# Autodesk Inventor assembly: Long Arm
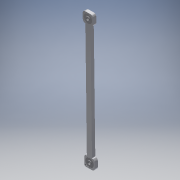
[picture p0: Inventor's stored thumbnail of the model, 180x180]
Saved by Autodesk Inventor 2016 (Build 200138000, 138)
## iProperties
Created: 2015-06-08
Part Number: Long Arm
Document SubType Name: Assembly
Designer: Dennis
Author: Dennis
## Documents named in this file (3)
- C:\Users\Dennis\Dropbox\NI Work\NI Slider Crank\Assemblies\Long Arm.iam
- C:\Users\Dennis\Dropbox\NI Work\NI Slider Crank\Parts\Arm Long.ipt
- C:\Users\Dennis\Dropbox\NI Work\NI Slider Crank\Parts\Bearing - 6384K342.ipt
## Components (3 placed, 2 different names)
1. Arm Long:1 — Mate:1, Mate:2, Mate:3, Mate:4
2. Bearing - 6384K342:1 — Mate:1, Mate:4
3. Bearing - 6384K342:2 — Mate:2, Mate:3
## Relationships (4: Mate 4)
- Mate:1: Arm Long:1 ↔ Bearing - 6384K342:1
- Mate:2: Arm Long:1 ↔ Bearing - 6384K342:2
- Mate:3: Arm Long:1 ↔ Bearing - 6384K342:2
- Mate:4: Arm Long:1 ↔ Bearing - 6384K342:1
